# Autodesk Inventor assembly: s-assy-motor-wrist3
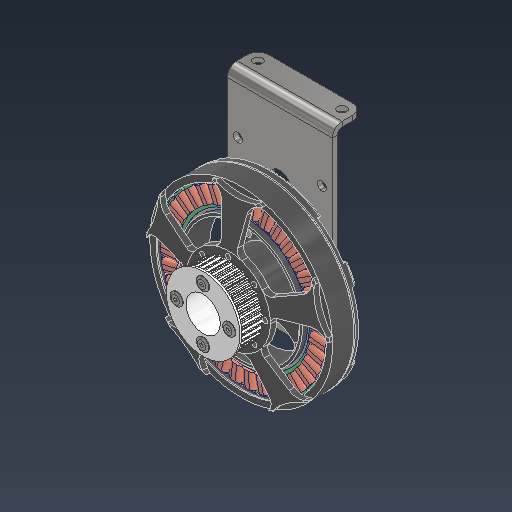
[picture p0: Inventor's stored thumbnail of the model, 512x512]
Saved by Autodesk Inventor 2021 (Build 250183000, 183)
## iProperties
Created: 2021-07-15
Part Number: s-assy-motor-wrist3
Document SubType Name: Assembly
Designer: yuta0
Author: yuta0
## Documents named in this file (8)
- C:\Users\yuta0\Documents\GitHub\catchrobo_hardware\assy-robot\s-assy-motor-wrist3.iam
- C:\Users\yuta0\Documents\GitHub\catchrobo_hardware\assy-robot\base12.ipt
- C:\Users\yuta0\Documents\GitHub\catchrobo_hardware\assy-robot\ex8108.iam
- C:\Users\yuta0\Documents\GitHub\catchrobo_hardware\assy-robot\CBSTNR3-16.ipt
- C:\Users\yuta0\Documents\GitHub\catchrobo_hardware\assy-robot\s-assy-unit-magnet.iam
- C:\Users\yuta0\Documents\GitHub\catchrobo_hardware\assy-robot\steel_plate5.ipt
- C:\Users\yuta0\Documents\GitHub\catchrobo_hardware\assy-robot\s-assy-unit-encoder.iam
- C:\Users\yuta0\Documents\GitHub\catchrobo_hardware\assy-robot\CB4-6.ipt
## Components (13 placed, 7 different names)
1. ex8108:1 [sub-assembly] — メイト:1, メイト:9, メイト:10, メイト:11, メイト:27, メイト:29, メイト:32, メイト:33, メイト:34
2. s-assy-unit-magnet:1 [sub-assembly] — メイト:9, メイト:10, メイト:11
3. steel_plate5:1 — メイト:27, メイト:28, メイト:29, メイト:30, メイト:31, メイト:37, メイト:38
4. s-assy-unit-encoder:1 [sub-assembly] — メイト:26, メイト:30, メイト:31
5. base12:1 — メイト:32, メイト:33, メイト:34, メイト:35, メイト:36
6. CBSTNR3-16:1 — メイト:35, メイト:36
7. CB4-6:1 — メイト:37, メイト:38
8. CBSTNR3-16:2
9. CB4-6:2
10. CBSTNR3-16:3
11. CB4-6:3
12. CBSTNR3-16:4
13. CB4-6:4
## Component patterns: (4 elements, first: CBSTNR3-16:1 + CB4-6:1)
## Relationships (17: Mate 17)
- メイト:1 [Mate]: ex8108:1
- メイト:9 [Mate]: ex8108:1 ↔ s-assy-unit-magnet:1
- メイト:10 [Mate]: ex8108:1 ↔ s-assy-unit-magnet:1
- メイト:11 [Mate]: ex8108:1 ↔ s-assy-unit-magnet:1
- メイト:26 [Mate]: s-assy-unit-encoder:1
- メイト:27 [Mate]: ex8108:1 ↔ steel_plate5:1
- メイト:28 [Mate]: steel_plate5:1
- メイト:29 [Mate]: ex8108:1 ↔ steel_plate5:1
- メイト:30 [Mate]: steel_plate5:1 ↔ s-assy-unit-encoder:1
- メイト:31 [Mate]: steel_plate5:1 ↔ s-assy-unit-encoder:1
- メイト:32 [Mate]: ex8108:1 ↔ base12:1
- メイト:33 [Mate]: ex8108:1 ↔ base12:1
- メイト:34 [Mate]: ex8108:1 ↔ base12:1
- メイト:35 [Mate]: base12:1 ↔ CBSTNR3-16:1
- メイト:36 [Mate]: base12:1 ↔ CBSTNR3-16:1
- メイト:37 [Mate]: steel_plate5:1 ↔ CB4-6:1
- メイト:38 [Mate]: steel_plate5:1 ↔ CB4-6:1
